# Autodesk Inventor assembly: Lens_mounted
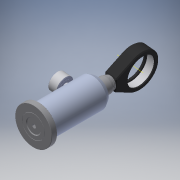
[picture p0: Inventor's stored thumbnail of the model, 180x180]
Saved by Autodesk Inventor 2016 (Build 200138000, 138)
## iProperties
Created: 2016-01-14
Part Number: Lens_mounted
Document SubType Name: Assembly
Designer: Conor Mow-Lowry
Author: Conor Mow-Lowry
## Documents named in this file (5)
- C:\Documents\Birmingham\Outreach\ThinkTank Michelson\Lens_mounted.iam
- C:\Documents\Birmingham\Outreach\ThinkTank Michelson\BE1_M-Step.ipt
- C:\Documents\Birmingham\Outreach\ThinkTank Michelson\PH50V_M-Step.ipt
- C:\Documents\Birmingham\Outreach\ThinkTank Michelson\TR50_M-Step.ipt
- C:\Documents\Birmingham\Outreach\ThinkTank Michelson\LMR1_M-Step.ipt
## Components (4 placed, 4 different names)
1. BE1_M-Step:1 — Mate:1, Mate:2, Mate:4, Angle:1
2. PH50V_M-Step:1 — Mate:1, Mate:2, Mate:3, Angle:1, Angle:2
3. TR50_M-Step:1 — Mate:3, Mate:4, Mate:5, Mate:6, Angle:2, Angle:3
4. LMR1_M-Step:1 — Mate:5, Mate:6, Angle:3
## Relationships (9: Mate 6, Angle 3)
- Mate:1: BE1_M-Step:1 ↔ PH50V_M-Step:1
- Mate:2: BE1_M-Step:1 ↔ PH50V_M-Step:1
- Mate:3: PH50V_M-Step:1 ↔ TR50_M-Step:1
- Mate:4 (-66 mm): BE1_M-Step:1 ↔ TR50_M-Step:1
- Mate:5: TR50_M-Step:1 ↔ LMR1_M-Step:1
- Mate:6: TR50_M-Step:1 ↔ LMR1_M-Step:1
- Angle:1 (0 deg): BE1_M-Step:1 ↔ PH50V_M-Step:1
- Angle:2 (0 deg): PH50V_M-Step:1 ↔ TR50_M-Step:1
- Angle:3 (0 deg): TR50_M-Step:1 ↔ LMR1_M-Step:1
